# Autodesk Inventor assembly: Functioning Test Chasis
(part 2 of 2)
- [Mate]: 1100x215 alum spacer 83062 K-S:14 ↔ Bearing Plate:4
- [Mate]: 10-32x1750_shcs_HX-SHCS 0.19-32x1.375x1-C:16 ↔ Bearing Plate:4
- [Mate]: 10-32 Nylock Nut:14 ↔ Motor Mount Plate Rev 2:4
- [Mate]: 1100x215 alum spacer 83062 K-S:15 ↔ Bearing Plate:4
- [Mate]: 10-32 Nylock Nut:16 ↔ Motor Mount Plate Rev 2:4
- [Mate]: 10-32x1750_shcs_HX-SHCS 0.19-32x1.375x1-C:13 ↔ Bearing Plate:4
- [Mate]: 10-32 Nylock Nut:13 ↔ 10-32x1750_shcs_HX-SHCS 0.19-32x1.375x1-C:13
- [Mate]: 10-32 Nylock Nut:13 ↔ Motor Mount Plate Rev 2:4
- [Mate]: 10-32x1750_shcs_HX-SHCS 0.19-32x1.375x1-C:13 ↔ Bearing Plate:4
- [Mate]: 1100x215 alum spacer 83062 K-S:13 ↔ 10-32x1750_shcs_HX-SHCS 0.19-32x1.375x1-C:13
- [Mate]: 1100x215 alum spacer 83062 K-S:13 ↔ Bearing Plate:4
- [Mate]: 10-32x1750_shcs_HX-SHCS 0.19-32x1.375x1-C:14 ↔ Bearing Plate:4
- [Mate]: 10-32x1750_shcs_HX-SHCS 0.19-32x1.375x1-C:14 ↔ Bearing Plate:4
- [Mate]: 1100x215 alum spacer 83062 K-S:16 ↔ 10-32x1750_shcs_HX-SHCS 0.19-32x1.375x1-C:14
- [Mate]: 1100x215 alum spacer 83062 K-S:16 ↔ Bearing Plate:4
- [Mate]: 10-32 Nylock Nut:15 ↔ Motor Mount Plate Rev 2:4
- [Mate]: CIM Motor SW:4 ↔ 10-32x0625_shcs_HX-SHCS 0.19-32x1.375x1-C:24
- [Mate]: Motor Mount Plate Rev 2:4 ↔ 10-32x0625_shcs_HX-SHCS 0.19-32x1.375x1-C:24
- [Mate]: Motor Mount Plate Rev 2:4 ↔ 10-32x0625_shcs_HX-SHCS 0.19-32x1.375x1-C:24
- [Mate]: CIM Motor SW:4 ↔ 10-32x0625_shcs_HX-SHCS 0.19-32x1.375x1-C:23
- [Mate]: Motor Mount Plate Rev 2:4 ↔ 10-32x0625_shcs_HX-SHCS 0.19-32x1.375x1-C:23
- [Mate]: Motor Mount Plate Rev 2:4 ↔ 10-32x0625_shcs_HX-SHCS 0.19-32x1.375x1-C:23
- [Mate]: 12T CIM Shaft:4 ↔ CIM Motor SW:4
- [Mate]: VEX 217-2736 0500 Collar Clamp:4 ↔ CIM Motor SW:4
- [Mate]: VEX 217-2736 0500 Collar Clamp:4 ↔ Motor Mount Plate Rev 2:4
- [Mate]: 12T CIM Shaft:4 ↔ CIM Motor SW:4
- [Mate]: CIM Motor SW:4 ↔ Motor Mount Plate Rev 2:4
- [Mate]: PG-71:4 ↔ 375 External Self Locking Ring_98430A134:4
- [Mate]: 48T 10mm bore gear:4 ↔ PG-71:4
- [Mate]: 10-32x1750_shcs_HX-SHCS 0.19-32x1.375x1-C:13 ↔ Motor Mount Plate Rev 2:4
- [Mate]: 10-32x1750_shcs_HX-SHCS 0.19-32x1.375x1-C:16 ↔ Motor Mount Plate Rev 2:4
- [Mate]: 1100x215 alum spacer 83062 K-S:13 ↔ Motor Mount Plate Rev 2:4
- [Mate]: PG-71:4 ↔ 438x406 spacer 13RS100043:4
- [Mate]: Motor Mount Plate Rev 2:4 ↔ 438x406 spacer 13RS100043:4
- [Mate]: Motor Mount Plate Rev 2:4 ↔ SHCS M4x10_91290A187:14
- [Mate]: Motor Mount Plate Rev 2:4 ↔ SHCS M4x10_91290A187:13
- [Mate]: Motor Mount Plate Rev 2:4 ↔ SHCS M4x10_91290A187:16
- [Mate]: Motor Mount Plate Rev 2:4 ↔ SHCS M4x10_91290A187:15
- [Mate]: Motor Mount Plate Rev 2:4 ↔ SHCS M4x10_91290A187:13
- [Mate]: Motor Mount Plate Rev 2:4 ↔ SHCS M4x10_91290A187:14
- [Mate]: Motor Mount Plate Rev 2:4 ↔ SHCS M4x10_91290A187:16
- [Mate]: Motor Mount Plate Rev 2:4 ↔ SHCS M4x10_91290A187:15
- [Mate]: PG-71:4 ↔ 438x406 spacer 13RS100043:4
- [Mate]: Motor Mount Plate Rev 2:4 ↔ PG-71:4
- [Mate]: 48T 10mm bore gear:4 ↔ 438x406 spacer 13RS100043:4
- [Mate]: PG-71:4 ↔ 375 External Self Locking Ring_98430A134:4
- [RelateRotation] (1 ul): 20t 1-25mod bevel gear:4 ↔ 40t 1-25mod bevel gear:4
- [Mate]: 20t 1-25mod bevel gear:4 ↔ Bevel Input Shaft:4
- [RelateRotation] (1 ul): 40T Sleeve Gear REV2:4 ↔ 48T 10mm bore gear:4
- [Mate]: 48T 10mm bore gear:4 ↔ PG-71:4
- [Mate]: 10-24 Hex Washer Rolling x 3-4_93882A213:24 ↔ 4 in HiGrip Wheel:4
- [Mate]: 10-24 Hex Washer Rolling x 3-4_93882A213:23 ↔ 4 in HiGrip Wheel:4
- [Mate]: 10-24 Hex Washer Rolling x 3-4_93882A213:22 ↔ 4 in HiGrip Wheel:4
- [Mate]: 375 Hex Hub:4 ↔ 4 in HiGrip Wheel:4
- [Mate]: 40t 1-25mod bevel gear:4 ↔ 4 in HiGrip Wheel:4
- Mate:505: Chasis:1 ↔ Motor Mount Plate Rev 2:3
- Flush:46: Chasis:1 ↔ Motor Mount Plate Rev 2:3
- Mate:506 (95.25 mm): Chasis:1 ↔ Motor Mount Plate Rev 2:3
- Mate:507: Chasis:1 ↔ Motor Mount Plate Rev 2:4
- Flush:47: Chasis:1 ↔ Motor Mount Plate Rev 2:4
- Mate:508 (95.25 mm): Chasis:1 ↔ Motor Mount Plate Rev 2:4
- [Mate]: 375 Hex Hub:5 ↔ 10-24 Hex Washer Rolling x 3-4_93882A213:30
- [Mate]: 375 Hex Hub:5 ↔ 10-24 Hex Washer Rolling x 3-4_93882A213:25
- [Mate]: 375 Hex Hub:5 ↔ 10-24 Hex Washer Rolling x 3-4_93882A213:29
- [Mate]: 375 Hex Hub:5 ↔ 10-24 Hex Washer Rolling x 3-4_93882A213:28
- [Mate]: 375 Hex Hub:5 ↔ 10-24 Hex Washer Rolling x 3-4_93882A213:27
- [Mate]: 375 Hex Hub:5 ↔ 10-24 Hex Washer Rolling x 3-4_93882A213:26
- [Mate]: 375 Hex Hub:5 ↔ 10-24 Hex Washer Rolling x 3-4_93882A213:26
- [Mate]: 375 Hex Hub:5 ↔ 10-24 Hex Washer Rolling x 3-4_93882A213:28
- [Mate]: 375 Hex Hub:5 ↔ 10-24 Hex Washer Rolling x 3-4_93882A213:27
- [Mate]: 375 Hex Hub:5 ↔ 10-24 Hex Washer Rolling x 3-4_93882A213:25
- [Mate]: 375 Hex Hub:5 ↔ 10-24 Hex Washer Rolling x 3-4_93882A213:30
- [Mate]: 375 Hex Hub:5 ↔ 10-24 Hex Washer Rolling x 3-4_93882A213:29
- [Mate]: 375 Hex Output Shaft Rev 2:5 ↔ 375 Hex Hub:5
- [Mate]: 375 Hex Output Shaft Rev 2:5 ↔ 375 Hex Hub:5
- [Mate]: FR6ZZ-L Hex Bearing:9 ↔ 375 Hex Output Shaft Rev 2:5
- [Mate]: FR6ZZ-L Hex Bearing:9 ↔ 375 Hex Output Shaft Rev 2:5
- [Mate]: 375 Hex Output Shaft Rev 2:5 ↔ 40t 1-25mod bevel gear:5
- [Mate]: 375 Hex Output Shaft Rev 2:5 ↔ 40t 1-25mod bevel gear:5
- [RevoluteJoint]: FR6ZZ-L Hex Bearing:10 ↔ AMS C Housing Rev 2:5
- [RevoluteJoint]: FR6ZZ-L Hex Bearing:9 ↔ AMS C Housing Rev 2:5
- [Mate]: FR6ZZ-L Hex Bearing:9 ↔ 125x443 spacer SPS-0750-0443-0125:5
- [Mate]: FR6ZZ-L Hex Bearing:9 ↔ 125x443 spacer SPS-0750-0443-0125:5
- [Mate]: 375 Hex Output Shaft Rev 2:5 ↔ 375 E-klip - Mcm 97431A320_97431A320:5
- [Mate]: 375 Hex Output Shaft Rev 2:5 ↔ 375 E-klip - Mcm 97431A320_97431A320:5
- [Mate]: 375 Hex Hub:5 ↔ 125x443 spacer SPS-0750-0443-0125:5
- [Flush]: FR6ZZ-L Hex Bearing:9 ↔ 375 Hex Output Shaft Rev 2:5
- [RevoluteJoint]: 10-32 Nylock Nut 1_90631A411:17 ↔ 10-32x1250_shcs:19
- [RevoluteJoint]: 10-32 Nylock Nut 1_90631A411:18 ↔ 10-32x1250_shcs:20
- [RevoluteJoint]: 10-32 Nylock Nut 1_90631A411:20 ↔ 10-32x1250_shcs:18
- [RevoluteJoint]: 10-32 Nylock Nut 1_90631A411:19 ↔ 10-32x1250_shcs:17
- [Mate]: 10-32x1250_shcs:18 ↔ Gear Plate:5
- [Mate]: 10-32x1250_shcs:18 ↔ 620x215 alum spacer 83062 K-S:18
- [Flush]: 10-32x1250_shcs:18 ↔ Gear Plate:5
- [Mate]: 620x215 alum spacer 83062 K-S:18 ↔ Gear Plate:5
- [Mate]: 10-32x1250_shcs:17 ↔ Gear Plate:5
- [Mate]: 10-32x1250_shcs:17 ↔ 620x215 alum spacer 83062 K-S:17
- [Flush]: 10-32x1250_shcs:17 ↔ Gear Plate:5
- [Mate]: 620x215 alum spacer 83062 K-S:17 ↔ Gear Plate:5
- [Mate]: 10-32x1250_shcs:19 ↔ Gear Plate:5
- [Flush]: 10-32x1250_shcs:19 ↔ Gear Plate:5
- [Mate]: 10-32x1250_shcs:19 ↔ 620x215 alum spacer 83062 K-S:19
- [Mate]: 620x215 alum spacer 83062 K-S:19 ↔ Gear Plate:5
- [Mate]: 10-32x1250_shcs:20 ↔ 620x215 alum spacer 83062 K-S:20
- [Flush]: 10-32x1250_shcs:20 ↔ Gear Plate:5
- [Mate]: 10-32x1250_shcs:20 ↔ Gear Plate:5
- [Mate]: 620x215 alum spacer 83062 K-S:20 ↔ Gear Plate:5
- [Mate]: FR8ZZ Bearing_smart:5 ↔ 12T CIM Shaft:5
- [Mate]: FR8ZZ Bearing_smart:5 ↔ 12T CIM Shaft:5
- [Mate]: 12T CIM Shaft:5 ↔ Gear Plate:5
- [Mate]: Bevel Input Shaft:5 ↔ FR6ZZ Bearing_smart:9
- [Mate]: Bevel Input Shaft:5 ↔ 500 Washer am-1001:9
- [Mate]: Bevel Input Shaft:5 ↔ 40T 20dp 375h_Inch - Spur gear 20DP 40T 14.5PA .372FW ---S40N3.0H2.0L0.25N:5
- [Mate]: Bevel Input Shaft:5 ↔ 40T 20dp 375h_Inch - Spur gear 20DP 40T 14.5PA .372FW ---S40N3.0H2.0L0.25N:5
- [Flush]: Bevel Input Shaft:5 ↔ 40T 20dp 375h_Inch - Spur gear 20DP 40T 14.5PA .372FW ---S40N3.0H2.0L0.25N:5
- [Mate]: Bevel Input Shaft:5 ↔ 500 Washer am-1001:10
- [Mate]: Bevel Input Shaft:5 ↔ FR6ZZ Bearing_smart:10
- [Mate]: 500 Washer am-1001:10 ↔ FR6ZZ Bearing_smart:10
- [Mate]: Bevel Input Shaft:5 ↔ 500 Washer am-1001:10
- [Flush]: Bevel Input Shaft:5 ↔ 500 Washer am-1001:9
- [Mate]: Gear Plate:5 ↔ FR6ZZ Bearing_smart:10
- [Mate]: Gear Plate:5 ↔ FR6ZZ Bearing_smart:10
- [RevoluteJoint]: 20t 1-25mod bevel gear:5 ↔ Bevel Input Shaft:5
- [Mate]: Gear Plate:5 ↔ 10-32x0625_shcs_HX-SHCS 0.19-32x1.375x1-C:27
- [Flush]: Gear Plate:5 ↔ 10-32x0625_shcs_HX-SHCS 0.19-32x1.375x1-C:27
- [Mate]: Gear Plate:5 ↔ 10-32x0625_shcs_HX-SHCS 0.19-32x1.375x1-C:26
- [Flush]: Gear Plate:5 ↔ 10-32x0625_shcs_HX-SHCS 0.19-32x1.375x1-C:26
- [Mate]: Gear Plate:5 ↔ 10-32x0625_shcs_HX-SHCS 0.19-32x1.375x1-C:25
- [Flush]: Gear Plate:5 ↔ 10-32x0625_shcs_HX-SHCS 0.19-32x1.375x1-C:25
- [Mate]: Gear Plate:5 ↔ 10-32x0625_shcs_HX-SHCS 0.19-32x1.375x1-C:28
- [Flush]: Gear Plate:5 ↔ 10-32x0625_shcs_HX-SHCS 0.19-32x1.375x1-C:28
- [Mate]: FR6ZZ Bearing_smart:9 ↔ 500 Washer am-1001:9
- [Mate]: AMS C Housing Rev 2:5 ↔ 10-32x1250_shcs:18
- [Mate]: AMS C Housing Rev 2:5 ↔ 10-32x1250_shcs:17
- [Mate]: AMS C Housing Rev 2:5 ↔ FR6ZZ Bearing_smart:9
- [Mate]: AMS C Housing Rev 2:5 ↔ FR8ZZ Bearing_smart:5
- [Mate]: 10-32x0625_shcs_HX-SHCS 0.19-32x1.375x1-C:27 ↔ 40T Sleeve Gear REV2:5
- [Mate]: 10-32x0625_shcs_HX-SHCS 0.19-32x1.375x1-C:28 ↔ 40T Sleeve Gear REV2:5
- [Mate]: 10-32x0625_shcs_HX-SHCS 0.19-32x1.375x1-C:25 ↔ 40T Sleeve Gear REV2:5
- [Mate]: 10-32x0625_shcs_HX-SHCS 0.19-32x1.375x1-C:26 ↔ 40T Sleeve Gear REV2:5
- [Mate]: 12T CIM Shaft:5 ↔ 40T Sleeve Gear REV2:5
- [Mate]: Gear Plate:5 ↔ 40T Sleeve Gear REV2:5
- [Mate]: 10-32 Nylock Nut:17 ↔ 10-32x1750_shcs_HX-SHCS 0.19-32x1.375x1-C:17
- [Mate]: 10-32x1750_shcs_HX-SHCS 0.19-32x1.375x1-C:20 ↔ 10-32 Nylock Nut:18
- [Mate]: 10-32x1750_shcs_HX-SHCS 0.19-32x1.375x1-C:19 ↔ 10-32 Nylock Nut:20
- [Mate]: 10-32x1750_shcs_HX-SHCS 0.19-32x1.375x1-C:18 ↔ 10-32 Nylock Nut:19
- [Mate]: 1100x215 alum spacer 83062 K-S:19 ↔ 10-32x1750_shcs_HX-SHCS 0.19-32x1.375x1-C:19
- [Mate]: 10-32x1750_shcs_HX-SHCS 0.19-32x1.375x1-C:19 ↔ Bearing Plate:5
- [Mate]: 10-32x1750_shcs_HX-SHCS 0.19-32x1.375x1-C:19 ↔ Bearing Plate:5
- [Mate]: 1100x215 alum spacer 83062 K-S:18 ↔ 10-32x1750_shcs_HX-SHCS 0.19-32x1.375x1-C:20
- [Mate]: 10-32x1750_shcs_HX-SHCS 0.19-32x1.375x1-C:20 ↔ Bearing Plate:5
- [Mate]: 1100x215 alum spacer 83062 K-S:18 ↔ Bearing Plate:5
- [Mate]: 10-32x1750_shcs_HX-SHCS 0.19-32x1.375x1-C:20 ↔ Bearing Plate:5
- [Mate]: 10-32 Nylock Nut:18 ↔ Motor Mount Plate Rev 2:5
- [Mate]: 1100x215 alum spacer 83062 K-S:19 ↔ Bearing Plate:5
- [Mate]: 10-32 Nylock Nut:20 ↔ Motor Mount Plate Rev 2:5
- [Mate]: 10-32x1750_shcs_HX-SHCS 0.19-32x1.375x1-C:17 ↔ Bearing Plate:5
- [Mate]: 10-32 Nylock Nut:17 ↔ 10-32x1750_shcs_HX-SHCS 0.19-32x1.375x1-C:17
- [Mate]: 10-32 Nylock Nut:17 ↔ Motor Mount Plate Rev 2:5
- [Mate]: 10-32x1750_shcs_HX-SHCS 0.19-32x1.375x1-C:17 ↔ Bearing Plate:5
- [Mate]: 1100x215 alum spacer 83062 K-S:17 ↔ 10-32x1750_shcs_HX-SHCS 0.19-32x1.375x1-C:17
- [Mate]: 1100x215 alum spacer 83062 K-S:17 ↔ Bearing Plate:5
- [Mate]: 10-32x1750_shcs_HX-SHCS 0.19-32x1.375x1-C:18 ↔ Bearing Plate:5
- [Mate]: 10-32x1750_shcs_HX-SHCS 0.19-32x1.375x1-C:18 ↔ Bearing Plate:5
- [Mate]: 1100x215 alum spacer 83062 K-S:20 ↔ 10-32x1750_shcs_HX-SHCS 0.19-32x1.375x1-C:18
- [Mate]: 1100x215 alum spacer 83062 K-S:20 ↔ Bearing Plate:5
- [Mate]: 10-32 Nylock Nut:19 ↔ Motor Mount Plate Rev 2:5
- [Mate]: CIM Motor SW:5 ↔ 10-32x0625_shcs_HX-SHCS 0.19-32x1.375x1-C:30
- [Mate]: Motor Mount Plate Rev 2:5 ↔ 10-32x0625_shcs_HX-SHCS 0.19-32x1.375x1-C:30
- [Mate]: Motor Mount Plate Rev 2:5 ↔ 10-32x0625_shcs_HX-SHCS 0.19-32x1.375x1-C:30
- [Mate]: CIM Motor SW:5 ↔ 10-32x0625_shcs_HX-SHCS 0.19-32x1.375x1-C:29
- [Mate]: Motor Mount Plate Rev 2:5 ↔ 10-32x0625_shcs_HX-SHCS 0.19-32x1.375x1-C:29
- [Mate]: Motor Mount Plate Rev 2:5 ↔ 10-32x0625_shcs_HX-SHCS 0.19-32x1.375x1-C:29
- [Mate]: 12T CIM Shaft:5 ↔ CIM Motor SW:5
- [Mate]: VEX 217-2736 0500 Collar Clamp:5 ↔ CIM Motor SW:5
- [Mate]: VEX 217-2736 0500 Collar Clamp:5 ↔ Motor Mount Plate Rev 2:5
- [Mate]: 12T CIM Shaft:5 ↔ CIM Motor SW:5
- [Mate]: CIM Motor SW:5 ↔ Motor Mount Plate Rev 2:5
- [Mate]: PG-71:5 ↔ 375 External Self Locking Ring_98430A134:5
- [Mate]: 48T 10mm bore gear:5 ↔ PG-71:5
- [Mate]: 10-32x1750_shcs_HX-SHCS 0.19-32x1.375x1-C:17 ↔ Motor Mount Plate Rev 2:5
- [Mate]: 10-32x1750_shcs_HX-SHCS 0.19-32x1.375x1-C:20 ↔ Motor Mount Plate Rev 2:5
- [Mate]: 1100x215 alum spacer 83062 K-S:17 ↔ Motor Mount Plate Rev 2:5
- [Mate]: PG-71:5 ↔ 438x406 spacer 13RS100043:5
- [Mate]: Motor Mount Plate Rev 2:5 ↔ 438x406 spacer 13RS100043:5
- [Mate]: Motor Mount Plate Rev 2:5 ↔ SHCS M4x10_91290A187:18
- [Mate]: Motor Mount Plate Rev 2:5 ↔ SHCS M4x10_91290A187:17
- [Mate]: Motor Mount Plate Rev 2:5 ↔ SHCS M4x10_91290A187:20
- [Mate]: Motor Mount Plate Rev 2:5 ↔ SHCS M4x10_91290A187:19
- [Mate]: Motor Mount Plate Rev 2:5 ↔ SHCS M4x10_91290A187:17
- [Mate]: Motor Mount Plate Rev 2:5 ↔ SHCS M4x10_91290A187:18
- [Mate]: Motor Mount Plate Rev 2:5 ↔ SHCS M4x10_91290A187:20
- [Mate]: Motor Mount Plate Rev 2:5 ↔ SHCS M4x10_91290A187:19
- [Mate]: PG-71:5 ↔ 438x406 spacer 13RS100043:5
- [Mate]: Motor Mount Plate Rev 2:5 ↔ PG-71:5
- [Mate]: 48T 10mm bore gear:5 ↔ 438x406 spacer 13RS100043:5
- [Mate]: PG-71:5 ↔ 375 External Self Locking Ring_98430A134:5
- [RelateRotation] (1 ul): 20t 1-25mod bevel gear:5 ↔ 40t 1-25mod bevel gear:5
- [Mate]: 20t 1-25mod bevel gear:5 ↔ Bevel Input Shaft:5
- [RelateRotation] (1 ul): 40T Sleeve Gear REV2:5 ↔ 48T 10mm bore gear:5
- [Mate]: 48T 10mm bore gear:5 ↔ PG-71:5
- [Mate]: 10-24 Hex Washer Rolling x 3-4_93882A213:30 ↔ 4 in HiGrip Wheel:5
- [Mate]: 10-24 Hex Washer Rolling x 3-4_93882A213:29 ↔ 4 in HiGrip Wheel:5
- [Mate]: 10-24 Hex Washer Rolling x 3-4_93882A213:28 ↔ 4 in HiGrip Wheel:5
- [Mate]: 375 Hex Hub:5 ↔ 4 in HiGrip Wheel:5
- [Mate]: 40t 1-25mod bevel gear:5 ↔ 4 in HiGrip Wheel:5
- Mate:634: Chasis:1 ↔ Motor Mount Plate Rev 2:5
- Flush:59: Chasis:1 ↔ Motor Mount Plate Rev 2:5
- Mate:635 (95.25 mm): Chasis:1 ↔ Motor Mount Plate Rev 2:5
## Named parameters: d170_d220 = 0 mm, d171_d221 = 0 mm, d174_d222 = 0 mm, d175_d223 = 0 mm, d176_d224 = 0 mm, d177_d225 = 0 mm, d178_d226 = 0 mm, d180_d227 = 0 mm, d181_d228 = 0 mm, d182_d229 = 0 mm, d183_d230 = 0 mm, d188_d231 = 0 mm, d189_d93_d166 = 0 mm, d193_d94_d167 = 0 mm, d196_d95_d168 = 0 mm, d205_d96_d169 = 0 mm, d208_d172 = 0 mm, d250_d173 = 0 mm, d251_d179 = 0 mm, d252_d184 = 0 mm, d260_d185 = 0 mm, d261_d186 = 0 mm, d265_d187 = 0 mm, d269_d190 = 0 mm, d281_d191 = 0 mm, d282_d192 = 0 mm, d283_d194 = 0 mm, d284_d195 = -120 deg, d285_d197 = 0 mm, d286_d198 = 0 mm, d287_d94_d139 = 0 mm, d288_d95_d140 = -154.263513 deg, d289_d96_d141 = 0 mm, d290_d97_d142 = 63.496867 deg, d291_d98_d143 = 0 mm, d292_d99_d144 = 150.286815 deg, d293_d100_d146 = 0 mm, d294_d101_d147 = 0 mm, d295_d102_d148 = 0 mm, d296_d103_d149 = 0 mm, d297_d104_d150 = 0 mm, d298_d122_d151 = 0 mm, d299_d123_d152 = 0 mm, d300_d124_d153 = 0 mm, d301_d125_d154 = 0 mm, d302_d126_d155 = 0 mm, d303_d127_d156 = 0 mm, d304_d128_d157 = 0 mm, d305_d129_d158 = 0 mm, d306_d130_d159 = 0 mm, d307_d131_d160 = 0 mm, d308_d132_d161 = 0 mm, d309_d133_d165 = 0 mm, d310_d102 = 0 mm, d311_d103 = 0 mm, d312_d104 = 0 mm, d313_d105 = 0 mm, d314_d106 = 0 mm, d315_d107 = 0 mm, d316_d108 = 0 mm, d317_d109 = 0 mm, d318_d110 = 0 mm, d319_d113 = 0 mm, d320_d114 = 0 mm, d321_d117 = 0 mm, d322_d118 = 74.365012 deg, d323_d119 = 0 mm, d324_d120 = 86.908841 deg, d325_d121 = 0 mm, d326_d122 = 0 mm, d327_d131 = 0 mm, d328_d132 = 0 mm, d329_d135 = 0 mm, d330_d136 = 0 mm, d331_d137 = 0 mm, d332_d138 = -163.765471 deg, d333_d95 = 0 mm, d334_d96 = 0 mm, d335_d97 = 0 mm, d336_d98 = 0 mm, d337_d99 = 0 mm, d338_d100 = 0 mm, d339_d101 = 0 mm, d340_d163 = 0 mm, d341_d126 = 0 mm, d342_d127 = 0 mm, d343_d128 = 0 mm, d344_d129 = 0 mm, d345_d162 = 0 mm, d346_d777 = 0 mm, d347_d778 = 1, d348_d776 = 1, d349_d263 = 0 mm, d350_d264 = 0 mm, d351_d266 = 0 mm, d352_d267 = 0 mm, d353_d268 = 0 mm, d354_d270 = 0 mm, d355_d271 = 0 mm, d356_d272 = 0 mm, d357_d273 = 0 mm, d358_d274 = 0 mm, d359_d275 = 0 mm, d360_d276 = 0 mm, d361_d277 = 0 mm, d362_d278 = 0 mm, d363_d279 = 0 mm, d364_d280 = 0 mm, d365_d232 = 0 mm, d366_d233 = 0 mm, d367_d234 = 0 mm, d368_d235 = 0 mm, d369_d236 = 0 mm, d370_d237 = 0 mm, d371_d238 = 0 mm, d372_d239 = 0 mm, d373_d240 = 0 mm, d374_d241 = 0 mm, d375_d242 = 0 mm, d376_d243 = 0 mm, d377_d244 = 0 mm, d378_d245 = 0 mm, d379_d246 = 0 mm, d380_d247 = 0 mm, d381_d248 = 0 mm, d383_d253 = 0 mm, d384_d254 = 0 mm, d385_d255 = 0 mm, d386_d256 = 0 mm, d387_d257 = 0 mm, d388_d258 = 0 mm, d389_d259 = 0 mm, d390_d262 = 0 mm, d391_d199 = 0 mm, d392_d200 = 0 mm, d393_d201 = 0 mm, d394_d202 = 0 mm, d395_d203 = 0 mm, d396_d204 = 0 mm, d397_d206 = 0 mm, d398_d207 = 0 mm, d399_d209 = 0 mm, d400_d210 = 0 mm, d401_d211 = 0 mm, d402_d212 = 0 mm, d403_d213 = 0 mm, d404_d214 = 0 mm, d405_d215 = 0 mm, d406_d216 = 0 mm, d407_d217 = 0 mm, d408_d218 = 0 mm, d409_d219 = 0 mm, d413_d291_d98_d143 = 0 mm, d414_d292_d99_d144 = 158.142554 deg, d415_d293_d100_d146 = 0 mm, d416_d294_d101_d147 = 0 mm, d417_d295_d102_d148 = 0 mm, d418_d296_d103_d149 = 0 mm, d419_d297_d104_d150 = 0 mm, d420_d298_d122_d151 = 0 mm, d421_d299_d123_d152 = 0 mm, d422_d300_d124_d153 = 0 mm, d423_d301_d125_d154 = 0 mm, d424_d302_d126_d155 = 0 mm, d425_d303_d127_d156 = 0 mm, d426_d304_d128_d157 = 0 mm, d427_d305_d129_d158 = 0 mm, d428_d306_d130_d159 = 0 mm, d429_d307_d131_d160 = 0 mm, d430_d308_d132_d161 = 0 mm, d431_d309_d133_d165 = 0 mm, d432_d310_d102 = 0 mm, d433_d311_d103 = 0 mm, d434_d312_d104 = 0 mm, d435_d313_d105 = 0 mm, d436_d314_d106 = 0 mm, d437_d315_d107 = 0 mm, d438_d316_d108 = 0 mm, d439_d317_d109 = 0 mm, d440_d318_d110 = 0 mm, d441_d319_d113 = 0 mm, d442_d320_d114 = 0 mm, d443_d321_d117 = 0 mm, d444_d322_d118 = 74.365055 deg, d445_d323_d119 = 0 mm, d446_d324_d120 = -44.871886 deg, d447_d325_d121 = 0 mm, d448_d326_d122 = 0 mm, d449_d327_d131 = 0 mm, d450_d328_d132 = 0 mm, d451_d329_d135 = 0 mm, d452_d330_d136 = 0 mm, d453_d331_d137 = 0 mm, d454_d332_d138 = 108.131962 deg, d455_d333_d95 = 0 mm, d456_d334_d96 = 0 mm, d457_d335_d97 = 0 mm, d458_d336_d98 = 0 mm, d459_d337_d99 = 0 mm, d460_d338_d100 = 0 mm, d461_d339_d101 = 0 mm, d462_d340_d163 = 0 mm, d463_d341_d126 = 0 mm, d464_d342_d127 = 0 mm, d465_d343_d128 = 0 mm, d466_d344_d129 = 0 mm, d467_d345_d162 = 0 mm, d468_d346_d777 = 0 mm, d469_d347_d778 = 1, d470_d348_d776 = 1, d471_d349_d263 = 0 mm, d472_d350_d264 = 0 mm, d473_d351_d266 = 0 mm, d474_d352_d267 = 0 mm, d475_d353_d268 = 0 mm, d476_d354_d270 = 0 mm, d477_d355_d271 = 0 mm, d478_d356_d272 = 0 mm, d479_d357_d273 = 0 mm, d480_d358_d274 = 0 mm, d481_d359_d275 = 0 mm, d482_d360_d276 = 0 mm, d483_d361_d277 = 0 mm, d484_d362_d278 = 0 mm, d485_d363_d279 = 0 mm, d486_d364_d280 = 0 mm, d487_d365_d232 = 0 mm, d488_d366_d233 = 0 mm, d489_d367_d234 = 0 mm, d490_d368_d235 = 0 mm, d491_d369_d236 = 0 mm, d492_d370_d237 = 0 mm, d493_d371_d238 = 0 mm, d494_d372_d239 = 0 mm, d495_d373_d240 = 0 mm, d496_d374_d241 = 0 mm, d497_d375_d242 = 0 mm, d498_d376_d243 = 0 mm, d499_d377_d244 = 0 mm, d500_d378_d245 = 0 mm, d501_d379_d246 = 0 mm, d502_d380_d247 = 0 mm, d503_d381_d248 = 0 mm, d504_d383_d253 = 0 mm, d505_d384_d254 = 0 mm, d506_d385_d255 = 0 mm, d507_d386_d256 = 0 mm, d508_d387_d257 = 0 mm, d509_d388_d258 = 0 mm, d510_d389_d259 = 0 mm, d511_d390_d262 = 0 mm, d512_d391_d199 = 0 mm, d513_d392_d200 = 0 mm, d514_d393_d201 = 0 mm, d515_d394_d202 = 0 mm, d516_d395_d203 = 0 mm, d517_d396_d204 = 0 mm, d518_d397_d206 = 0 mm, d519_d398_d207 = 0 mm, d520_d399_d209 = 0 mm, d521_d400_d210 = 0 mm, d522_d401_d211 = 0 mm, d523_d402_d212 = 0 mm, d524_d403_d213 = 0 mm, d525_d404_d214 = 0 mm, d526_d405_d215 = 0 mm, d527_d406_d216 = 0 mm, d528_d407_d217 = 0 mm, d529_d408_d218 = 0 mm, d530_d409_d219 = 0 mm, d531_d170_d220 = 0 mm, d532_d171_d221 = 0 mm, d533_d174_d222 = 0 mm, d534_d175_d223 = 0 mm, d535_d176_d224 = 0 mm, d536_d177_d225 = 0 mm, d537_d178_d226 = 0 mm, d538_d180_d227 = 0 mm, d539_d181_d228 = 0 mm, d540_d182_d229 = 0 mm, d541_d183_d230 = 0 mm, d542_d188_d231 = 0 mm, d543_d189_d93_d166 = 0 mm, d544_d193_d94_d167 = 0 mm, d545_d196_d95_d168 = 0 mm, d546_d205_d96_d169 = 0 mm, d547_d208_d172 = 0 mm, d548_d250_d173 = 0 mm, d549_d251_d179 = 0 mm, d550_d252_d184 = 0 mm, d551_d260_d185 = 0 mm, d552_d261_d186 = 0 mm, d553_d265_d187 = 0 mm, d554_d269_d190 = 0 mm, d555_d281_d191 = 0 mm, d556_d282_d192 = 0 mm, d557_d283_d194 = 0 mm, d558_d284_d195 = -120 deg, d559_d285_d197 = 0 mm, d560_d286_d198 = 0 mm, d561_d287_d94_d139 = 0 mm, d562_d288_d95_d140 = 144.106003 deg, d563_d289_d96_d141 = 0 mm, d564_d290_d97_d142 = -119.943795 deg, d565_d413_d291_d98_d143 = 0 mm, d566_d414_d292_d99_d144 = -34.983371 deg, d567_d415_d293_d100_d146 = 0 mm, d568_d416_d294_d101_d147 = 0 mm, d569_d417_d295_d102_d148 = 0 mm, d570_d418_d296_d103_d149 = 0 mm, d571_d419_d297_d104_d150 = 0 mm, d572_d420_d298_d122_d151 = 0 mm, d573_d421_d299_d123_d152 = 0 mm, d574_d422_d300_d124_d153 = 0 mm, d575_d423_d301_d125_d154 = 0 mm, d576_d424_d302_d126_d155 = 0 mm, d577_d425_d303_d127_d156 = 0 mm, d578_d426_d304_d128_d157 = 0 mm, d579_d427_d305_d129_d158 = 0 mm, d580_d428_d306_d130_d159 = 0 mm, d581_d429_d307_d131_d160 = 0 mm, d582_d430_d308_d132_d161 = 0 mm, d583_d431_d309_d133_d165 = 0 mm, d584_d432_d310_d102 = 0 mm, d585_d433_d311_d103 = 0 mm, d586_d434_d312_d104 = 0 mm, d587_d435_d313_d105 = 0 mm, d588_d436_d314_d106 = 0 mm, d589_d437_d315_d107 = 0 mm, d590_d438_d316_d108 = 0 mm, d591_d439_d317_d109 = 0 mm, d592_d440_d318_d110 = 0 mm, d593_d441_d319_d113 = 0 mm, d594_d442_d320_d114 = 0 mm, d595_d443_d321_d117 = 0 mm, d596_d444_d322_d118 = 74.365067 deg, d597_d445_d323_d119 = 0 mm, d598_d446_d324_d120 = 29.518133 deg, d599_d447_d325_d121 = 0 mm, d600_d448_d326_d122 = 0 mm, d601_d449_d327_d131 = 0 mm, d602_d450_d328_d132 = 0 mm, d603_d451_d329_d135 = 0 mm, d604_d452_d330_d136 = 0 mm, d605_d453_d331_d137 = 0 mm, d606_d454_d332_d138 = 154.802613 deg, d607_d455_d333_d95 = 0 mm, d608_d456_d334_d96 = 0 mm, d609_d457_d335_d97 = 0 mm, d610_d458_d336_d98 = 0 mm, d611_d459_d337_d99 = 0 mm, d612_d460_d338_d100 = 0 mm, d613_d461_d339_d101 = 0 mm, d614_d462_d340_d163 = 0 mm, d615_d463_d341_d126 = 0 mm, d616_d464_d342_d127 = 0 mm, d617_d465_d343_d128 = 0 mm, d618_d466_d344_d129 = 0 mm, d619_d467_d345_d162 = 0 mm, d620_d468_d346_d777 = 0 mm, d621_d469_d347_d778 = 1, d622_d470_d348_d776 = 1, d623_d471_d349_d263 = 0 mm, d624_d472_d350_d264 = 0 mm, d625_d473_d351_d266 = 0 mm, d626_d474_d352_d267 = 0 mm, d627_d475_d353_d268 = 0 mm, d628_d476_d354_d270 = 0 mm, d629_d477_d355_d271 = 0 mm, d630_d478_d356_d272 = 0 mm, d631_d479_d357_d273 = 0 mm, d632_d480_d358_d274 = 0 mm, d633_d481_d359_d275 = 0 mm, d634_d482_d360_d276 = 0 mm, d635_d483_d361_d277 = 0 mm, d636_d484_d362_d278 = 0 mm, d637_d485_d363_d279 = 0 mm, d638_d486_d364_d280 = 0 mm, d639_d487_d365_d232 = 0 mm, d640_d488_d366_d233 = 0 mm, d641_d489_d367_d234 = 0 mm, d642_d490_d368_d235 = 0 mm, d643_d491_d369_d236 = 0 mm, d644_d492_d370_d237 = 0 mm, d645_d493_d371_d238 = 0 mm, d646_d494_d372_d239 = 0 mm, d647_d495_d373_d240 = 0 mm, d648_d496_d374_d241 = 0 mm, d649_d497_d375_d242 = 0 mm, d650_d498_d376_d243 = 0 mm, d651_d499_d377_d244 = 0 mm, d652_d500_d378_d245 = 0 mm, d653_d501_d379_d246 = 0 mm, d654_d502_d380_d247 = 0 mm, d655_d503_d381_d248 = 0 mm, d656_d504_d383_d253 = 0 mm, d657_d505_d384_d254 = 0 mm, d658_d506_d385_d255 = 0 mm, d659_d507_d386_d256 = 0 mm, d660_d508_d387_d257 = 0 mm, d661_d509_d388_d258 = 0 mm, d662_d510_d389_d259 = 0 mm, d663_d511_d390_d262 = 0 mm, d664_d512_d391_d199 = 0 mm, d665_d513_d392_d200 = 0 mm, d666_d514_d393_d201 = 0 mm, d667_d515_d394_d202 = 0 mm, d668_d516_d395_d203 = 0 mm, d669_d517_d396_d204 = 0 mm, d670_d518_d397_d206 = 0 mm, d671_d519_d398_d207 = 0 mm, d672_d520_d399_d209 = 0 mm, d673_d521_d400_d210 = 0 mm, d674_d522_d401_d211 = 0 mm, d675_d523_d402_d212 = 0 mm, d676_d524_d403_d213 = 0 mm, d677_d525_d404_d214 = 0 mm, d678_d526_d405_d215 = 0 mm, d679_d527_d406_d216 = 0 mm, d680_d528_d407_d217 = 0 mm, d681_d529_d408_d218 = 0 mm, d682_d530_d409_d219 = 0 mm, d683_d531_d170_d220 = 0 mm, d684_d532_d171_d221 = 0 mm, d685_d533_d174_d222 = 0 mm, d686_d534_d175_d223 = 0 mm, d687_d535_d176_d224 = 0 mm, d688_d536_d177_d225 = 0 mm, d689_d537_d178_d226 = 0 mm, d690_d538_d180_d227 = 0 mm, d691_d539_d181_d228 = 0 mm, d692_d540_d182_d229 = 0 mm, d693_d541_d183_d230 = 0 mm, d694_d542_d188_d231 = 0 mm, d695_d543_d189_d93_d166 = 0 mm, d696_d544_d193_d94_d167 = 0 mm, d697_d545_d196_d95_d168 = 0 mm, d698_d546_d205_d96_d169 = 0 mm, d699_d547_d208_d172 = 0 mm, d700_d548_d250_d173 = 0 mm, d701_d549_d251_d179 = 0 mm, d702_d550_d252_d184 = 0 mm, d703_d551_d260_d185 = 0 mm, d704_d552_d261_d186 = 0 mm, d705_d553_d265_d187 = 0 mm, d706_d554_d269_d190 = 0 mm, d707_d555_d281_d191 = 0 mm, d708_d556_d282_d192 = 0 mm, d709_d557_d283_d194 = 0 mm, d710_d558_d284_d195 = -120 deg, d711_d559_d285_d197 = 0 mm, d712_d560_d286_d198 = 0 mm, d713_d561_d287_d94_d139 = 0 mm, d714_d562_d288_d95_d140 = 160.838145 deg, d715_d563_d289_d96_d141 = 0 mm, d716_d564_d290_d97_d142 = -57.222776 deg, d723_d413_d291_d98_d143 = 0 mm, d724_d414_d292_d99_d144 = 108.226383 deg, d725_d415_d293_d100_d146 = 0 mm, d726_d416_d294_d101_d147 = 0 mm, d727_d417_d295_d102_d148 = 0 mm, d728_d418_d296_d103_d149 = 0 mm, d729_d419_d297_d104_d150 = 0 mm, d730_d420_d298_d122_d151 = 0 mm, d731_d421_d299_d123_d152 = 0 mm, d732_d422_d300_d124_d153 = 0 mm, d733_d423_d301_d125_d154 = 0 mm, d734_d424_d302_d126_d155 = 0 mm, d735_d425_d303_d127_d156 = 0 mm, d736_d426_d304_d128_d157 = 0 mm, d737_d427_d305_d129_d158 = 0 mm, d738_d428_d306_d130_d159 = 0 mm, d739_d429_d307_d131_d160 = 0 mm, d740_d430_d308_d132_d161 = 0 mm, d741_d431_d309_d133_d165 = 0 mm, d742_d432_d310_d102 = 0 mm, d743_d433_d311_d103 = 0 mm, d744_d434_d312_d104 = 0 mm, d745_d435_d313_d105 = 0 mm, d746_d436_d314_d106 = 0 mm, d747_d437_d315_d107 = 0 mm, d748_d438_d316_d108 = 0 mm, d749_d439_d317_d109 = 0 mm, d750_d440_d318_d110 = 0 mm, d751_d441_d319_d113 = 0 mm, d752_d442_d320_d114 = 0 mm, d753_d443_d321_d117 = 0 mm, d754_d444_d322_d118 = 74.365047 deg, d755_d445_d323_d119 = 0 mm, d756_d446_d324_d120 = -10.131945 deg, d757_d447_d325_d121 = 0 mm, d758_d448_d326_d122 = 0 mm, d759_d449_d327_d131 = 0 mm, d760_d450_d328_d132 = 0 mm, d761_d451_d329_d135 = 0 mm, d762_d452_d330_d136 = 0 mm, d763_d453_d331_d137 = 0 mm, d764_d454_d332_d138 = 29.377487 deg, d765_d455_d333_d95 = 0 mm, d766_d456_d334_d96 = 0 mm, d767_d457_d335_d97 = 0 mm, d768_d458_d336_d98 = 0 mm, d769_d459_d337_d99 = 0 mm, d770_d460_d338_d100 = 0 mm, d771_d461_d339_d101 = 0 mm, d772_d462_d340_d163 = 0 mm, d773_d463_d341_d126 = 0 mm, d774_d464_d342_d127 = 0 mm, d775_d465_d343_d128 = 0 mm, d776_d466_d344_d129 = 0 mm, d777_d467_d345_d162 = 0 mm, d778_d468_d346_d777 = 0 mm, d779_d469_d347_d778 = 1, d780_d470_d348_d776 = 1, d781_d471_d349_d263 = 0 mm, d782_d472_d350_d264 = 0 mm, d783_d473_d351_d266 = 0 mm, d784_d474_d352_d267 = 0 mm, d785_d475_d353_d268 = 0 mm, d786_d476_d354_d270 = 0 mm, d787_d477_d355_d271 = 0 mm, d788_d478_d356_d272 = 0 mm, d789_d479_d357_d273 = 0 mm, d790_d480_d358_d274 = 0 mm, d791_d481_d359_d275 = 0 mm, d792_d482_d360_d276 = 0 mm, d793_d483_d361_d277 = 0 mm, d794_d484_d362_d278 = 0 mm, d795_d485_d363_d279 = 0 mm, d796_d486_d364_d280 = 0 mm, d797_d487_d365_d232 = 0 mm, d798_d488_d366_d233 = 0 mm, d799_d489_d367_d234 = 0 mm, d800_d490_d368_d235 = 0 mm, d801_d491_d369_d236 = 0 mm, d802_d492_d370_d237 = 0 mm, d803_d493_d371_d238 = 0 mm, d804_d494_d372_d239 = 0 mm, d805_d495_d373_d240 = 0 mm, d806_d496_d374_d241 = 0 mm, d807_d497_d375_d242 = 0 mm, d808_d498_d376_d243 = 0 mm, d809_d499_d377_d244 = 0 mm, d810_d500_d378_d245 = 0 mm, d811_d501_d379_d246 = 0 mm, d812_d502_d380_d247 = 0 mm, d813_d503_d381_d248 = 0 mm, d814_d504_d383_d253 = 0 mm, d815_d505_d384_d254 = 0 mm, d816_d506_d385_d255 = 0 mm, d817_d507_d386_d256 = 0 mm, d818_d508_d387_d257 = 0 mm, d819_d509_d388_d258 = 0 mm, d820_d510_d389_d259 = 0 mm, d821_d511_d390_d262 = 0 mm, d822_d512_d391_d199 = 0 mm, d823_d513_d392_d200 = 0 mm, d824_d514_d393_d201 = 0 mm, d825_d515_d394_d202 = 0 mm, d826_d516_d395_d203 = 0 mm, d827_d517_d396_d204 = 0 mm, d828_d518_d397_d206 = 0 mm, d829_d519_d398_d207 = 0 mm, d830_d520_d399_d209 = 0 mm, d831_d521_d400_d210 = 0 mm, d832_d522_d401_d211 = 0 mm, d833_d523_d402_d212 = 0 mm, d834_d524_d403_d213 = 0 mm, d835_d525_d404_d214 = 0 mm, d836_d526_d405_d215 = 0 mm, d837_d527_d406_d216 = 0 mm, d838_d528_d407_d217 = 0 mm, d839_d529_d408_d218 = 0 mm, d840_d530_d409_d219 = 0 mm, d841_d531_d170_d220 = 0 mm, d842_d532_d171_d221 = 0 mm, d843_d533_d174_d222 = 0 mm, d844_d534_d175_d223 = 0 mm, d845_d535_d176_d224 = 0 mm, d846_d536_d177_d225 = 0 mm, d847_d537_d178_d226 = 0 mm, d848_d538_d180_d227 = 0 mm, d849_d539_d181_d228 = 0 mm, d850_d540_d182_d229 = 0 mm, d851_d541_d183_d230 = 0 mm, d852_d542_d188_d231 = 0 mm, d853_d543_d189_d93_d166 = 0 mm, d854_d544_d193_d94_d167 = 0 mm, d855_d545_d196_d95_d168 = 0 mm, d856_d546_d205_d96_d169 = 0 mm, d857_d547_d208_d172 = 0 mm, d858_d548_d250_d173 = 0 mm, d859_d549_d251_d179 = 0 mm, d860_d550_d252_d184 = 0 mm, d861_d551_d260_d185 = 0 mm, d862_d552_d261_d186 = 0 mm, d863_d553_d265_d187 = 0 mm, d864_d554_d269_d190 = 0 mm, d865_d555_d281_d191 = 0 mm, d866_d556_d282_d192 = 0 mm, d867_d557_d283_d194 = 0 mm, d868_d558_d284_d195 = -120 deg, d869_d559_d285_d197 = 0 mm, d870_d560_d286_d198 = 0 mm, d871_d561_d287_d94_d139 = 0 mm, d872_d562_d288_d95_d140 = 119.00231 deg, d873_d563_d289_d96_d141 = 0 mm, d874_d564_d290_d97_d142 = 179.464536 deg
